# Autodesk Inventor assembly: A8-9000
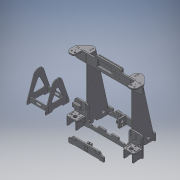
[picture p0: Inventor's stored thumbnail of the model, 180x180]
Saved by Autodesk Inventor 2016 SP2 (Build 200236200, 236)
## iProperties
Created: 2017-04-26
Part Number: A8-9000
Document SubType Name: Assembly
Designer: EV
Author: EV
## Documents named in this file (18)
- E:\Inventor Projects\ANET A8\A8-9000.iam
- E:\Inventor Projects\ANET A8\A8-0010.ipt
- E:\Inventor Projects\ANET A8\A8-0012.ipt
- E:\Inventor Projects\ANET A8\A8-0011.ipt
- E:\Inventor Projects\ANET A8\A8-0004.ipt
- E:\Inventor Projects\ANET A8\A8-0009.ipt
- E:\Inventor Projects\ANET A8\A8-0003.ipt
- E:\Inventor Projects\ANET A8\A8-0017.ipt
- E:\Inventor Projects\ANET A8\A8-0018.ipt
- E:\Inventor Projects\ANET A8\A8-0008.ipt
- E:\Inventor Projects\ANET A8\A8-0013.ipt
- E:\Inventor Projects\ANET A8\A8-0014.ipt
- E:\Inventor Projects\ANET A8\A8-0001.ipt
- E:\Inventor Projects\ANET A8\A8-0002.ipt
- E:\Inventor Projects\ANET A8\A8-0016.ipt
- E:\Inventor Projects\ANET A8\A8-0005.ipt
- E:\Inventor Projects\ANET A8\A8-0007.ipt
- E:\Inventor Projects\ANET A8\A8-0006.ipt
## Components (30 placed, 17 different names)
1. A8-0010:1 — Flush:1, Flush:2, Mate:1, Mate:2, Mate:3, Mate:4, Mate:5, Flush:3, Flush:4, Flush:5, Flush:6, Flush:9, Mate:11, Angle:1, Flush:12, Flush:21, Flush:22, Mate:24, Mate:25, Mate:26, Mate:27, Mate:28, Mate:29, Mate:30, Mate:31, Mate:33, Mate:35, Mate:36, Mate:37, Angle:3, Flush:34
2. A8-0012:1 — Mate:2, Mate:4, Flush:4, Mate:6, Mate:8, Mate:12
3. A8-0012:2 — Mate:3, Mate:5, Flush:3, Mate:10
4. A8-0011:1 — Flush:5, Flush:6, Mate:6, Mate:7, Flush:7, Mate:9, Flush:8, Rigid:5
5. A8-0004:1 — Mate:7, Mate:8, Flush:7
6. A8-0004:2 — Mate:9, Mate:10, Flush:8
7. A8-0009:1 — Flush:9, Mate:11, Mate:12, Mate:13, Mate:14, Flush:10, Mate:15, Flush:11, Mate:16, Mate:17, Mate:18, Mate:19, Rigid:3, Rigid:4
8. A8-0003:1 — Mate:13, Mate:14, Flush:10
9. A8-0017:1 — Mate:15, Flush:11, Mate:16
10. A8-0018:1 — Mate:17, Mate:18, Angle:1, Mate:19
11. A8-0008:1 — Flush:12, Flush:21, Flush:22, Mate:20, Mate:21, Mate:22, Angle:2, Mate:23, Rigid:1, Rigid:2
12. A8-0013:1 — Mate:20, Mate:21, Mate:22, Angle:2, Flush:23, Flush:25
13. A8-0013:2 — Flush:23, Flush:25, Mate:23
14. A8-0014:1 — Rigid:1
15. A8-0014:2 — Rigid:2
16. A8-0014:3 — Rigid:3
17. A8-0014:4 — Rigid:4
18. A8-0001:1 — Flush:26, Flush:28, Mate:24, Mate:25, Mate:26, Flush:29, Mate:32
19. A8-0001:2 — Flush:26, Flush:28, Mate:27
20. A8-0001:3 — Mate:28, Flush:29, Mate:29, Flush:30, Flush:32
21. A8-0001:4 — Flush:30, Flush:32, Mate:30, Mate:34
22. A8-0002:1 — Mate:31, Mate:32, Mate:33, Flush:33
23. A8-0002:2 — Flush:33, Mate:34, Mate:35
24. A8-0016:1 — Mate:36, Mate:37, Angle:3, Flush:34, Flush:35, Flush:37, Mate:38
25. A8-0016:2 — Flush:35, Flush:37, Mate:38
26. A8-0005:1 — Rigid:5
27. A8-0007:1 — Mate:39, Flush:38, Mate:40, Flush:39, Flush:41, Mate:41, Mate:42, Angle:4, Mate:43, Mate:45
28. A8-0007:2 — Flush:39, Flush:41, Mate:44
29. A8-0006:1 — Mate:41, Mate:42, Angle:4, Mate:43, Flush:42, Flush:44, Mate:44
30. A8-0006:2 — Flush:42, Flush:44, Mate:45
## Relationships (84: Mate 45, Flush 30, WeldJoint 5, Angle 4)
- Flush:1: A8-0010:1
- Flush:2: A8-0010:1
- Mate:1: A8-0010:1
- Mate:2: A8-0010:1 ↔ A8-0012:1
- Mate:3: A8-0010:1 ↔ A8-0012:2
- Mate:4: A8-0010:1 ↔ A8-0012:1
- Mate:5: A8-0010:1 ↔ A8-0012:2
- Flush:3: A8-0010:1 ↔ A8-0012:2
- Flush:4: A8-0010:1 ↔ A8-0012:1
- Flush:5: A8-0010:1 ↔ A8-0011:1
- Flush:6: A8-0010:1 ↔ A8-0011:1
- Mate:6: A8-0012:1 ↔ A8-0011:1
- Mate:7: A8-0011:1 ↔ A8-0004:1
- Mate:8: A8-0012:1 ↔ A8-0004:1
- Flush:7: A8-0011:1 ↔ A8-0004:1
- Mate:9: A8-0011:1 ↔ A8-0004:2
- Mate:10: A8-0012:2 ↔ A8-0004:2
- Flush:8: A8-0011:1 ↔ A8-0004:2
- Flush:9: A8-0010:1 ↔ A8-0009:1
- Mate:11: A8-0010:1 ↔ A8-0009:1
- Mate:12: A8-0012:1 ↔ A8-0009:1
- Mate:13: A8-0009:1 ↔ A8-0003:1
- Mate:14: A8-0009:1 ↔ A8-0003:1
- Flush:10: A8-0009:1 ↔ A8-0003:1
- Mate:15: A8-0009:1 ↔ A8-0017:1
- Flush:11: A8-0009:1 ↔ A8-0017:1
- Mate:16: A8-0009:1 ↔ A8-0017:1
- Mate:17: A8-0009:1 ↔ A8-0018:1
- Mate:18: A8-0009:1 ↔ A8-0018:1
- Angle:1 (180 deg): A8-0010:1 ↔ A8-0018:1
- Mate:19: A8-0009:1 ↔ A8-0018:1
- Flush:12: A8-0010:1 ↔ A8-0008:1
- Flush:21: A8-0010:1 ↔ A8-0008:1
- Flush:22 (-150 mm): A8-0010:1 ↔ A8-0008:1
- Mate:20: A8-0008:1 ↔ A8-0013:1
- Mate:21: A8-0008:1 ↔ A8-0013:1
- Mate:22: A8-0008:1 ↔ A8-0013:1
- Angle:2 (180 deg): A8-0008:1 ↔ A8-0013:1
- Flush:23: A8-0013:1 ↔ A8-0013:2
- Flush:25: A8-0013:1 ↔ A8-0013:2
- Mate:23: A8-0008:1 ↔ A8-0013:2
- Rigid:1 [WeldJoint]: A8-0008:1 ↔ A8-0014:1
- Rigid:2 [WeldJoint]: A8-0008:1 ↔ A8-0014:2
- Rigid:3 [WeldJoint]: A8-0009:1 ↔ A8-0014:3
- Rigid:4 [WeldJoint]: A8-0009:1 ↔ A8-0014:4
- Flush:26: A8-0001:1 ↔ A8-0001:2
- Flush:28: A8-0001:1 ↔ A8-0001:2
- Mate:24: A8-0010:1 ↔ A8-0001:1
- Mate:25: A8-0010:1 ↔ A8-0001:1
- Mate:26: A8-0010:1 ↔ A8-0001:1
- Mate:27: A8-0010:1 ↔ A8-0001:2
- Mate:28: A8-0010:1 ↔ A8-0001:3
- Flush:29: A8-0001:1 ↔ A8-0001:3
- Mate:29: A8-0010:1 ↔ A8-0001:3
- Flush:30: A8-0001:3 ↔ A8-0001:4
- Flush:32: A8-0001:3 ↔ A8-0001:4
- Mate:30: A8-0010:1 ↔ A8-0001:4
- Mate:31: A8-0010:1 ↔ A8-0002:1
- Mate:32: A8-0001:1 ↔ A8-0002:1
- Mate:33: A8-0010:1 ↔ A8-0002:1
- Flush:33: A8-0002:1 ↔ A8-0002:2
- Mate:34: A8-0001:4 ↔ A8-0002:2
- Mate:35: A8-0010:1 ↔ A8-0002:2
- Mate:36: A8-0010:1 ↔ A8-0016:1
- Mate:37 (-7.5 mm): A8-0010:1 ↔ A8-0016:1
- Angle:3 (0 deg): A8-0010:1 ↔ A8-0016:1
- Flush:34 (25 mm): A8-0010:1 ↔ A8-0016:1
- Flush:35: A8-0016:1 ↔ A8-0016:2
- Flush:37: A8-0016:1 ↔ A8-0016:2
- Mate:38: A8-0016:1 ↔ A8-0016:2
- Rigid:5 [WeldJoint] (-10 mm): A8-0011:1 ↔ A8-0005:1
- Mate:39: A8-0007:1
- Flush:38: A8-0007:1
- Mate:40 (-350 mm): A8-0007:1
- Flush:39: A8-0007:1 ↔ A8-0007:2
- Flush:41: A8-0007:1 ↔ A8-0007:2
- Mate:41: A8-0007:1 ↔ A8-0006:1
- Mate:42: A8-0007:1 ↔ A8-0006:1
- Angle:4 (0 deg): A8-0007:1 ↔ A8-0006:1
- Mate:43: A8-0007:1 ↔ A8-0006:1
- Flush:42: A8-0006:1 ↔ A8-0006:2
- Flush:44: A8-0006:1 ↔ A8-0006:2
- Mate:44: A8-0007:2 ↔ A8-0006:1
- Mate:45: A8-0007:1 ↔ A8-0006:2
